# Autodesk Inventor assembly: Drive Assembly
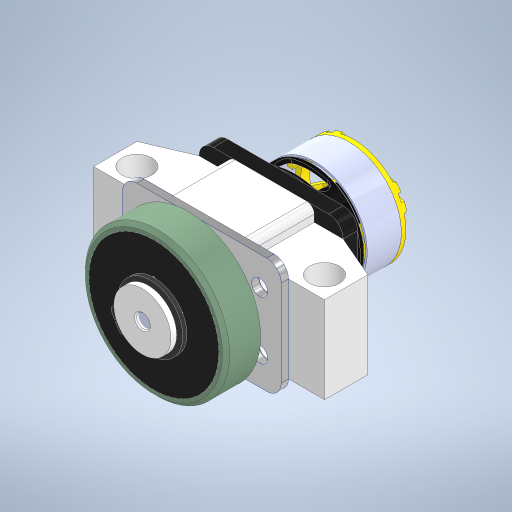
[picture p0: Inventor's stored thumbnail of the model, 512x512]
Saved by Autodesk Inventor 2023.2 (Build 272271000, 271)
## iProperties
Created: 2023-04-12
Part Number: Drive Assembly
Document SubType Name: Assembly
Designer: Nathan Cai
Mass: 34.861 g
Surface Area: 143.766 cm^2
Volume: 13.0781 cm^3
Density: 2.66561 g/cm^3
Author: Nathan Cai
## Documents named in this file (6)
- C:\Users\Nathan Cai\Documents\Inventor\Flatbread V1.0\Drive Assembly.iam
- C:\Users\Nathan Cai\Documents\Inventor\Flatbread V1.0\Custom Wheel V2.0\Recessed Wheels V2.0.iam
- C:\Users\Nathan Cai\Documents\Inventor\Flatbread V1.0\Motor Sleeve.ipt
- C:\Users\Nathan Cai\Documents\Inventor\Flatbread V1.0\RR Brushless\RR-Brushless-Planetary.iam
- C:\Users\Nathan Cai\Documents\Inventor\Flatbread V1.0\Motor Plates - Rear Insert.ipt
- C:\Users\Nathan Cai\Documents\Inventor\Flatbread V1.0\Motor Plates.ipt
## Components (5 placed, 5 different names)
1. Recessed Wheels V2.0:1 [sub-assembly] — Mate:4, Mate:5
2. Motor Sleeve:1 — Mate:1, Flush:1, Mate:3, Mate:7, Mate:8, Mate:9
3. RR-Brushless-Planetary:1 [sub-assembly] — Mate:1, Flush:1, Mate:2, Mate:4, Mate:5, Mate:6
4. Motor Plates - Rear Insert:1 — Mate:2, Mate:3, Mate:7
5. Motor Plates:1 — Mate:6, Mate:8, Mate:9
## Relationships (10: Mate 9, Flush 1)
- Mate:1: Motor Sleeve:1 ↔ RR-Brushless-Planetary:1
- Flush:1: Motor Sleeve:1 ↔ RR-Brushless-Planetary:1
- Mate:2: RR-Brushless-Planetary:1 ↔ Motor Plates - Rear Insert:1
- Mate:3: Motor Sleeve:1 ↔ Motor Plates - Rear Insert:1
- Mate:4: Recessed Wheels V2.0:1 ↔ RR-Brushless-Planetary:1
- Mate:5: Recessed Wheels V2.0:1 ↔ RR-Brushless-Planetary:1
- Mate:6: RR-Brushless-Planetary:1 ↔ Motor Plates:1
- Mate:7: Motor Sleeve:1 ↔ Motor Plates - Rear Insert:1
- Mate:8: Motor Sleeve:1 ↔ Motor Plates:1
- Mate:9: Motor Sleeve:1 ↔ Motor Plates:1
